# Autodesk Inventor assembly: Сборка
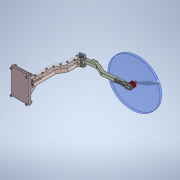
[picture p0: Inventor's stored thumbnail of the model, 180x180]
Saved by Autodesk Inventor 2021.2 (Build 252289000, 289)
## iProperties
Created: 2024-10-29
Part Number: Сборка
Document SubType Name: Assembly
Designer: barko
Author: barko
## Documents named in this file (27)
- C:\Users\DELL\Desktop\Personal\PID_controller\PID_controller\Mechanics\3D_model\Сборка.iam
- C:\Users\DELL\Desktop\Personal\PID_controller\PID_controller\Mechanics\3D_model\Детали твёрдого тела\Ножка 1.ipt
- C:\Users\DELL\Desktop\Personal\PID_controller\PID_controller\Mechanics\3D_model\Детали твёрдого тела\Ножка 2.ipt
- C:\Users\DELL\Desktop\Personal\PID_controller\PID_controller\Mechanics\3D_model\Детали твёрдого тела\Скобка 1.ipt
- C:\Users\DELL\Desktop\Personal\PID_controller\PID_controller\Mechanics\3D_model\Детали твёрдого тела\Скобка 2.ipt
- C:\Users\DELL\Desktop\Personal\PID_controller\PID_controller\Mechanics\3D_model\Детали твёрдого тела\Фланец.ipt
- C:\Users\DELL\Desktop\Personal\PID_controller\PID_controller\Mechanics\3D_model\Детали твёрдого тела\Луч.ipt
- C:\Users\DELL\Desktop\Personal\PID_controller\PID_controller\Mechanics\3D_model\Детали твёрдого тела\Ложечка.ipt
- C:\Users\DELL\Desktop\Personal\PID_controller\PID_controller\Mechanics\3D_model\Моторчик.ipt
- C:\Users\DELL\Desktop\Personal\PID_controller\PID_controller\Mechanics\3D_model\Пропеллер.ipt
- C:\Users\DELL\Documents\Inventor\Content Center Files\R2021\ru-RU\Nut GOST 15524-70\Гайка M4-6H ГОСТ 15524-70.ipt
- C:\Users\DELL\Documents\Inventor\Content Center Files\R2021\ru-RU\GOST 11738-84\Винт M4-6gx20 ГОСТ 11738-84.ipt
- C:\Users\DELL\Desktop\Personal\PID_controller\PID_controller\Mechanics\3D_model\Подшипник.ipt
- C:\Users\DELL\Documents\Inventor\Content Center Files\R2021\ru-RU\GOST 5915-70\Гайка M6-6H ГОСТ 5915-70(1).ipt
- C:\Users\DELL\Documents\Inventor\Content Center Files\R2021\ru-RU\GOST 11738-84\Винт M6-6gx50 ГОСТ 11738-84.ipt
- C:\Users\DELL\Documents\Inventor\Content Center Files\R2021\ru-RU\GOST 11738-84\Винт M6-6gx25 ГОСТ 11738-84.ipt
- C:\Users\DELL\Documents\Inventor\Content Center Files\R2021\ru-RU\GOST 11371-78  A\Шайба 6 ГОСТ 11371-78.ipt
- C:\Users\DELL\Documents\Inventor\Content Center Files\R2021\ru-RU\Washer 1 GOST 6402-78\Шайба 6Л ГОСТ 6402-78.ipt
- C:\Users\DELL\Documents\Inventor\Content Center Files\R2021\ru-RU\GOST 17475-80 (2)\Винт 2.M6-6gx30 ГОСТ 17475-80.ipt
- C:\Users\DELL\Documents\Inventor\Content Center Files\R2021\ru-RU\ISO 10642(1)\ISO 10642 - M3x8.ipt
- C:\Users\DELL\Documents\Inventor\Content Center Files\R2021\ru-RU\ISO 10642(1)\ISO 10642 - M3x12.ipt
- C:\Users\DELL\Desktop\Personal\PID_controller\PID_controller\Mechanics\3D_model\Детали твёрдого тела\Вал стержень.ipt
- C:\Users\DELL\Desktop\Personal\PID_controller\PID_controller\Mechanics\3D_model\Детали твёрдого тела\Вал насадка 1.ipt
- C:\Users\DELL\Desktop\Personal\PID_controller\PID_controller\Mechanics\3D_model\Метизы\Гайка M4-6H ГОСТ 11860-85.ipt
- C:\Users\DELL\Desktop\Personal\PID_controller\PID_controller\Mechanics\3D_model\Метизы\Шайба A 4 ГОСТ 6958-78.ipt
- C:\Users\DELL\Desktop\Personal\PID_controller\PID_controller\Mechanics\3D_model\Метизы\DIN 912 - M4 x 0,7 x 35 x 20.ipt
- C:\Users\DELL\Documents\Inventor\Content Center Files\R2021\ru-RU\GOST 5916-70\Гайка M4-6H ГОСТ 5916-70.ipt
## Components (71 placed, 26 different names)
1. Ножка 1:1 — Совмещение:1, Угол:1, Совмещение:16, Совмещение:18, Совмещение:20, Совмещение:22, Совмещение:24, Совмещение:26, Совмещение:28, Совмещение:46, Совмещение:58, Совмещение:62, Совмещение:64
2. Ножка 2:1 — Совмещение:17, Совмещение:19, Совмещение:21, Совмещение:23, Совмещение:25, Совмещение:27, Совмещение:29, Совмещение:59, Совмещение:60, Совмещение:63, Совмещение:65
3. Скобка 1:1 — Совмещение:42, Совмещение:43, Совмещение:44, Совмещение:53, Совмещение:54, Совмещение:55
4. Скобка 2:1 — Совмещение:47, Совмещение:48, Совмещение:49, Совмещение:50, Совмещение:51, Совмещение:52
5. Фланец:1 — Совмещение:66, Совмещение:67, Совмещение:68, Совмещение:69, Совмещение:70, Совмещение:71, Совмещение:72, Совмещение:73, Совмещение:74, Совмещение:75, Совмещение:76, Совмещение:77, Вставка:6, Вставка:7, Вставка:8, Вставка:9, Заподлицо:2, Заподлицо:3, Заподлицо:4, Заподлицо:5
6. Луч:1 — Заподлицо:1, Совмещение:1, Угол:1, Совмещение:37, Совмещение:38, Совмещение:40, Совмещение:41, Совмещение:96, Угол:2, Совмещение:97, Заподлицо:6, Совмещение:104, Заподлицо:7
7. Ложечка:1 — Совмещение:87, Совмещение:88, Совмещение:91, Совмещение:92, Совмещение:93, Совмещение:94, Совмещение:96, Угол:2, Совмещение:97, Заподлицо:6, Совмещение:98, Совмещение:99
8. Моторчик:1 — Вставка:2, Совмещение:98, Совмещение:99
9. Пропеллер:1 — Вставка:2
10. Подшипник:1 — Вставка:21
11. Подшипник:2 — Вставка:20, Вставка:24
12. Вал стержень:1 — Совмещение:104, Заподлицо:7
13. Вал насадка 1:1 — Вставка:20
14. Гайка M4-6H ГОСТ 11860-85:1 — Вставка:22
15. Шайба A 4 ГОСТ 6958-78:1 — Вставка:21, Вставка:22
16. Гайка M4-6H ГОСТ 11860-85:2
17. Шайба A 4 ГОСТ 6958-78:2 — Вставка:24
18. DIN 912 - M4 x 0,7 x 35 x 20:1
19. Гайка ГОСТ 5916-70 M4:1 — Совмещение:16, Совмещение:17
20. DIN 912 - M4 x 0,7 x 35 x 20:2
21. DIN 912 - M4 x 0,7 x 35 x 20:3
22. DIN 912 - M4 x 0,7 x 35 x 20:4
23. DIN 912 - M4 x 0,7 x 35 x 20:5
24. DIN 912 - M4 x 0,7 x 35 x 20:6
25. DIN 912 - M4 x 0,7 x 35 x 20:7
26. Гайка ГОСТ 5916-70 M4:2 — Совмещение:18, Совмещение:19
27. Гайка ГОСТ 5916-70 M4:3 — Совмещение:20, Совмещение:21
28. Гайка ГОСТ 5916-70 M4:4 — Совмещение:22, Совмещение:23
29. Гайка ГОСТ 5916-70 M4:5 — Совмещение:24, Совмещение:25
30. Гайка ГОСТ 5916-70 M4:6 — Совмещение:26, Совмещение:27
31. Гайка ГОСТ 5916-70 M4:7 — Совмещение:28, Совмещение:29
32. Винт ГОСТ 11738-84 M 4x20:1 — Совмещение:45, Совмещение:46
33. Гайка ГОСТ 15524-70 M4:1 — Совмещение:42, Совмещение:43, Совмещение:44, Совмещение:45
34. Винт ГОСТ 11738-84 M 4x20:5 — Совмещение:37, Совмещение:39
35. Гайка ГОСТ 15524-70 M4:2 — Совмещение:38, Совмещение:39, Совмещение:40, Совмещение:41
36. Винт ГОСТ 11738-84 M 4x20:2 — Совмещение:56, Совмещение:58
37. Винт ГОСТ 11738-84 M 4x20:3 — Совмещение:60, Совмещение:61
38. Винт ГОСТ 11738-84 M 4x20:4 — Совмещение:57, Совмещение:59
39. Гайка ГОСТ 15524-70 M4:3 — Совмещение:47, Совмещение:48, Совмещение:49, Совмещение:61
40. Гайка ГОСТ 15524-70 M4:4 — Совмещение:53, Совмещение:54, Совмещение:55, Совмещение:56
41. Гайка ГОСТ 15524-70 M4:5 — Совмещение:50, Совмещение:51, Совмещение:52, Совмещение:57
42. Гайка ГОСТ 5915-70 M6:1 — Совмещение:69, Совмещение:72, Совмещение:73, Совмещение:80
43. Гайка ГОСТ 5915-70 M6:2 — Совмещение:71, Совмещение:74, Совмещение:75, Совмещение:81
44. Гайка ГОСТ 5915-70 M6:3 — Совмещение:70, Совмещение:76, Совмещение:77, Совмещение:79
45. Гайка ГОСТ 5915-70 M6:4 — Совмещение:66, Совмещение:67, Совмещение:68, Совмещение:78
46. Винт ГОСТ 11738-84 M 6x50:1 — Совмещение:64, Совмещение:79
47. Винт ГОСТ 11738-84 M 6x25:2 — Совмещение:63, Совмещение:80
48. Винт ГОСТ 11738-84 M 6x25:1 — Совмещение:62, Совмещение:78
49. Винт ГОСТ 11738-84 M 6x50:2 — Совмещение:65, Совмещение:81
50. Шайба  ГОСТ 11371-78 6,4:1 — Вставка:6, Вставка:10
51. Шайба  ГОСТ 11371-78 6,4:2 — Вставка:7, Вставка:11
52. Шайба  ГОСТ 11371-78 6,4:3 — Вставка:8, Вставка:13
53. Шайба  ГОСТ 11371-78 6,4:4 — Вставка:9, Вставка:12
54. Шайба 1 ГОСТ 6402-78 6Л:1 — Вставка:10, Вставка:16
55. Шайба 1 ГОСТ 6402-78 6Л:2 — Вставка:11, Вставка:15
56. Шайба 1 ГОСТ 6402-78 6Л:3 — Вставка:12, Вставка:17
57. Шайба 1 ГОСТ 6402-78 6Л:4 — Вставка:13, Вставка:14
58. Гайка ГОСТ 5915-70 M6:5 — Вставка:14, Совмещение:85
59. Гайка ГОСТ 5915-70 M6:6 — Вставка:15, Совмещение:84
60. Гайка ГОСТ 5915-70 M6:7 — Вставка:16, Совмещение:82
61. Гайка ГОСТ 5915-70 M6:8 — Вставка:17, Совмещение:83
62. Винт 2 ГОСТ 17475-80 M6 x 30:1 — Совмещение:82, Заподлицо:3
63. Винт 2 ГОСТ 17475-80 M6 x 30:2 — Совмещение:83, Заподлицо:2
64. Винт 2 ГОСТ 17475-80 M6 x 30:3 — Совмещение:85, Заподлицо:5
65. Винт 2 ГОСТ 17475-80 M6 x 30:4 — Совмещение:84, Заподлицо:4
66. ISO 10642 M3x12:2 — Совмещение:87
67. ISO 10642 M3x12:3 — Совмещение:88
68. ISO 10642 M3x8:1 — Совмещение:91
69. ISO 10642 M3x8:2 — Совмещение:92
70. ISO 10642 M3x8:3 — Совмещение:93
71. ISO 10642 M3x8:4 — Совмещение:94
## Relationships (116: Mate 89, Insert 18, Flush 7, Angle 2)
- Вставка:2 [Insert] (2 mm): Моторчик:1 ↔ Пропеллер:1
- Заподлицо:1 [Flush]: Луч:1
- Совмещение:1 [Mate]: Ножка 1:1 ↔ Луч:1
- Угол:1 [Angle] (0 deg): Ножка 1:1 ↔ Луч:1
- [Mate]: Ножка 1:1 ↔ DIN 912 - M4 x 0,7 x 35 x 20:1
- [Mate]: Ножка 1:1 ↔ DIN 912 - M4 x 0,7 x 35 x 20:1
- [Mate]: Ножка 1:1 ↔ DIN 912 - M4 x 0,7 x 35 x 20:2
- [Mate]: Ножка 1:1 ↔ DIN 912 - M4 x 0,7 x 35 x 20:2
- [Mate]: Ножка 1:1 ↔ DIN 912 - M4 x 0,7 x 35 x 20:3
- [Mate]: Ножка 1:1 ↔ DIN 912 - M4 x 0,7 x 35 x 20:3
- [Mate]: Ножка 1:1 ↔ DIN 912 - M4 x 0,7 x 35 x 20:4
- [Mate]: Ножка 1:1 ↔ DIN 912 - M4 x 0,7 x 35 x 20:4
- [Mate]: Ножка 1:1 ↔ DIN 912 - M4 x 0,7 x 35 x 20:5
- [Mate]: Ножка 1:1 ↔ DIN 912 - M4 x 0,7 x 35 x 20:5
- [Mate]: Ножка 1:1 ↔ DIN 912 - M4 x 0,7 x 35 x 20:6
- [Mate]: Ножка 1:1 ↔ DIN 912 - M4 x 0,7 x 35 x 20:6
- [Mate]: Ножка 1:1 ↔ DIN 912 - M4 x 0,7 x 35 x 20:7
- [Mate]: Ножка 1:1 ↔ DIN 912 - M4 x 0,7 x 35 x 20:7
- Совмещение:16 [Mate]: Ножка 1:1 ↔ Гайка ГОСТ 5916-70 M4:1
- Совмещение:17 [Mate]: Ножка 2:1 ↔ Гайка ГОСТ 5916-70 M4:1
- Совмещение:18 [Mate]: Ножка 1:1 ↔ Гайка ГОСТ 5916-70 M4:2
- Совмещение:19 [Mate]: Ножка 2:1 ↔ Гайка ГОСТ 5916-70 M4:2
- Совмещение:20 [Mate]: Ножка 1:1 ↔ Гайка ГОСТ 5916-70 M4:3
- Совмещение:21 [Mate]: Ножка 2:1 ↔ Гайка ГОСТ 5916-70 M4:3
- Совмещение:22 [Mate]: Ножка 1:1 ↔ Гайка ГОСТ 5916-70 M4:4
- Совмещение:23 [Mate]: Ножка 2:1 ↔ Гайка ГОСТ 5916-70 M4:4
- Совмещение:24 [Mate]: Ножка 1:1 ↔ Гайка ГОСТ 5916-70 M4:5
- Совмещение:25 [Mate]: Ножка 2:1 ↔ Гайка ГОСТ 5916-70 M4:5
- Совмещение:26 [Mate]: Ножка 1:1 ↔ Гайка ГОСТ 5916-70 M4:6
- Совмещение:27 [Mate]: Ножка 2:1 ↔ Гайка ГОСТ 5916-70 M4:6
- Совмещение:28 [Mate]: Ножка 1:1 ↔ Гайка ГОСТ 5916-70 M4:7
- Совмещение:29 [Mate]: Ножка 2:1 ↔ Гайка ГОСТ 5916-70 M4:7
- Совмещение:37 [Mate]: Луч:1 ↔ Винт ГОСТ 11738-84 M 4x20:5
- Совмещение:38 [Mate]: Луч:1 ↔ Гайка ГОСТ 15524-70 M4:2
- Совмещение:39 [Mate]: Винт ГОСТ 11738-84 M 4x20:5 ↔ Гайка ГОСТ 15524-70 M4:2
- Совмещение:40 [Mate]: Луч:1 ↔ Гайка ГОСТ 15524-70 M4:2
- Совмещение:41 [Mate]: Луч:1 ↔ Гайка ГОСТ 15524-70 M4:2
- Совмещение:42 [Mate]: Скобка 1:1 ↔ Гайка ГОСТ 15524-70 M4:1
- Совмещение:43 [Mate]: Скобка 1:1 ↔ Гайка ГОСТ 15524-70 M4:1
- Совмещение:44 [Mate]: Скобка 1:1 ↔ Гайка ГОСТ 15524-70 M4:1
- Совмещение:45 [Mate]: Винт ГОСТ 11738-84 M 4x20:1 ↔ Гайка ГОСТ 15524-70 M4:1
- Совмещение:46 [Mate]: Ножка 1:1 ↔ Винт ГОСТ 11738-84 M 4x20:1
- Совмещение:47 [Mate]: Скобка 2:1 ↔ Гайка ГОСТ 15524-70 M4:3
- Совмещение:48 [Mate]: Скобка 2:1 ↔ Гайка ГОСТ 15524-70 M4:3
- Совмещение:49 [Mate]: Скобка 2:1 ↔ Гайка ГОСТ 15524-70 M4:3
- Совмещение:50 [Mate]: Скобка 2:1 ↔ Гайка ГОСТ 15524-70 M4:5
- Совмещение:51 [Mate]: Скобка 2:1 ↔ Гайка ГОСТ 15524-70 M4:5
- Совмещение:52 [Mate]: Скобка 2:1 ↔ Гайка ГОСТ 15524-70 M4:5
- Совмещение:53 [Mate]: Скобка 1:1 ↔ Гайка ГОСТ 15524-70 M4:4
- Совмещение:54 [Mate]: Скобка 1:1 ↔ Гайка ГОСТ 15524-70 M4:4
- Совмещение:55 [Mate]: Скобка 1:1 ↔ Гайка ГОСТ 15524-70 M4:4
- Совмещение:56 [Mate]: Винт ГОСТ 11738-84 M 4x20:2 ↔ Гайка ГОСТ 15524-70 M4:4
- Совмещение:57 [Mate]: Винт ГОСТ 11738-84 M 4x20:4 ↔ Гайка ГОСТ 15524-70 M4:5
- Совмещение:58 [Mate]: Ножка 1:1 ↔ Винт ГОСТ 11738-84 M 4x20:2
- Совмещение:59 [Mate]: Ножка 2:1 ↔ Винт ГОСТ 11738-84 M 4x20:4
- Совмещение:60 [Mate]: Ножка 2:1 ↔ Винт ГОСТ 11738-84 M 4x20:3
- Совмещение:61 [Mate]: Винт ГОСТ 11738-84 M 4x20:3 ↔ Гайка ГОСТ 15524-70 M4:3
- Совмещение:62 [Mate]: Ножка 1:1 ↔ Винт ГОСТ 11738-84 M 6x25:1
- Совмещение:63 [Mate]: Ножка 2:1 ↔ Винт ГОСТ 11738-84 M 6x25:2
- Совмещение:64 [Mate]: Ножка 1:1 ↔ Винт ГОСТ 11738-84 M 6x50:1
- Совмещение:65 [Mate]: Ножка 2:1 ↔ Винт ГОСТ 11738-84 M 6x50:2
- Совмещение:66 [Mate]: Фланец:1 ↔ Гайка ГОСТ 5915-70 M6:4
- Совмещение:67 [Mate]: Фланец:1 ↔ Гайка ГОСТ 5915-70 M6:4
- Совмещение:68 [Mate]: Фланец:1 ↔ Гайка ГОСТ 5915-70 M6:4
- Совмещение:69 [Mate]: Фланец:1 ↔ Гайка ГОСТ 5915-70 M6:1
- Совмещение:70 [Mate]: Фланец:1 ↔ Гайка ГОСТ 5915-70 M6:3
- Совмещение:71 [Mate]: Фланец:1 ↔ Гайка ГОСТ 5915-70 M6:2
- Совмещение:72 [Mate]: Фланец:1 ↔ Гайка ГОСТ 5915-70 M6:1
- Совмещение:73 [Mate]: Фланец:1 ↔ Гайка ГОСТ 5915-70 M6:1
- Совмещение:74 [Mate]: Фланец:1 ↔ Гайка ГОСТ 5915-70 M6:2
- Совмещение:75 [Mate]: Фланец:1 ↔ Гайка ГОСТ 5915-70 M6:2
- Совмещение:76 [Mate]: Фланец:1 ↔ Гайка ГОСТ 5915-70 M6:3
- Совмещение:77 [Mate]: Фланец:1 ↔ Гайка ГОСТ 5915-70 M6:3
- Совмещение:78 [Mate]: Гайка ГОСТ 5915-70 M6:4 ↔ Винт ГОСТ 11738-84 M 6x25:1
- Совмещение:79 [Mate]: Гайка ГОСТ 5915-70 M6:3 ↔ Винт ГОСТ 11738-84 M 6x50:1
- Совмещение:80 [Mate]: Гайка ГОСТ 5915-70 M6:1 ↔ Винт ГОСТ 11738-84 M 6x25:2
- Совмещение:81 [Mate]: Гайка ГОСТ 5915-70 M6:2 ↔ Винт ГОСТ 11738-84 M 6x50:2
- Вставка:6 [Insert]: Фланец:1 ↔ Шайба  ГОСТ 11371-78 6,4:1
- Вставка:7 [Insert]: Фланец:1 ↔ Шайба  ГОСТ 11371-78 6,4:2
- Вставка:8 [Insert]: Фланец:1 ↔ Шайба  ГОСТ 11371-78 6,4:3
- Вставка:9 [Insert]: Фланец:1 ↔ Шайба  ГОСТ 11371-78 6,4:4
- Вставка:10 [Insert]: Шайба  ГОСТ 11371-78 6,4:1 ↔ Шайба 1 ГОСТ 6402-78 6Л:1
- Вставка:11 [Insert]: Шайба  ГОСТ 11371-78 6,4:2 ↔ Шайба 1 ГОСТ 6402-78 6Л:2
- Вставка:12 [Insert]: Шайба  ГОСТ 11371-78 6,4:4 ↔ Шайба 1 ГОСТ 6402-78 6Л:3
- Вставка:13 [Insert]: Шайба  ГОСТ 11371-78 6,4:3 ↔ Шайба 1 ГОСТ 6402-78 6Л:4
- Вставка:14 [Insert]: Шайба 1 ГОСТ 6402-78 6Л:4 ↔ Гайка ГОСТ 5915-70 M6:5
- Вставка:15 [Insert]: Шайба 1 ГОСТ 6402-78 6Л:2 ↔ Гайка ГОСТ 5915-70 M6:6
- Вставка:16 [Insert]: Шайба 1 ГОСТ 6402-78 6Л:1 ↔ Гайка ГОСТ 5915-70 M6:7
- Вставка:17 [Insert]: Шайба 1 ГОСТ 6402-78 6Л:3 ↔ Гайка ГОСТ 5915-70 M6:8
- Совмещение:82 [Mate]: Гайка ГОСТ 5915-70 M6:7 ↔ Винт 2 ГОСТ 17475-80 M6 x 30:1
- Совмещение:83 [Mate]: Гайка ГОСТ 5915-70 M6:8 ↔ Винт 2 ГОСТ 17475-80 M6 x 30:2
- Совмещение:84 [Mate]: Гайка ГОСТ 5915-70 M6:6 ↔ Винт 2 ГОСТ 17475-80 M6 x 30:4
- Совмещение:85 [Mate]: Гайка ГОСТ 5915-70 M6:5 ↔ Винт 2 ГОСТ 17475-80 M6 x 30:3
- Заподлицо:2 [Flush] (9 mm): Фланец:1 ↔ Винт 2 ГОСТ 17475-80 M6 x 30:2
- Заподлицо:3 [Flush] (9 mm): Фланец:1 ↔ Винт 2 ГОСТ 17475-80 M6 x 30:1
- Заподлицо:4 [Flush] (9 mm): Фланец:1 ↔ Винт 2 ГОСТ 17475-80 M6 x 30:4
- Заподлицо:5 [Flush] (9 mm): Фланец:1 ↔ Винт 2 ГОСТ 17475-80 M6 x 30:3
- Совмещение:87 [Mate]: Ложечка:1 ↔ ISO 10642 M3x12:2
- Совмещение:88 [Mate]: Ложечка:1 ↔ ISO 10642 M3x12:3
- Совмещение:91 [Mate]: Ложечка:1 ↔ ISO 10642 M3x8:1
- Совмещение:92 [Mate]: Ложечка:1 ↔ ISO 10642 M3x8:2
- Совмещение:93 [Mate]: Ложечка:1 ↔ ISO 10642 M3x8:3
- Совмещение:94 [Mate]: Ложечка:1 ↔ ISO 10642 M3x8:4
- Совмещение:96 [Mate]: Луч:1 ↔ Ложечка:1
- Угол:2 [Angle] (180 deg): Луч:1 ↔ Ложечка:1
- Совмещение:97 [Mate]: Луч:1 ↔ Ложечка:1
- Заподлицо:6 [Flush]: Луч:1 ↔ Ложечка:1
- Совмещение:98 [Mate]: Ложечка:1 ↔ Моторчик:1
- Совмещение:99 [Mate]: Ложечка:1 ↔ Моторчик:1
- Совмещение:104 [Mate]: Луч:1 ↔ Вал стержень:1
- Заподлицо:7 [Flush]: Луч:1 ↔ Вал стержень:1
- Вставка:20 [Insert]: Подшипник:2 ↔ Вал насадка 1:1
- Вставка:21 [Insert]: Подшипник:1 ↔ Шайба A 4 ГОСТ 6958-78:1
- Вставка:22 [Insert]: Гайка M4-6H ГОСТ 11860-85:1 ↔ Шайба A 4 ГОСТ 6958-78:1
- [Insert]: Гайка M4-6H ГОСТ 11860-85:2 ↔ Шайба A 4 ГОСТ 6958-78:2
- Вставка:24 [Insert]: Подшипник:2 ↔ Шайба A 4 ГОСТ 6958-78:2
## Named parameters: d207_d206 = 0 mm
